# Autodesk Inventor assembly: SensorAssembly_v2
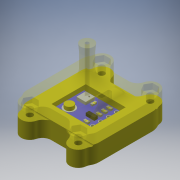
[picture p0: Inventor's stored thumbnail of the model, 180x180]
Saved by Autodesk Inventor 2018 (Build 220112000, 112)
## iProperties
Created: 2020-03-10
Part Number: SensorAssembly_v2
Document SubType Name: Assembly
Designer: Ivan
Author: Ivan
## Documents named in this file (4)
- C:\Users\Ivan\Documents\GitHub\IdealGas\3D Model\SensorAssembly_v2.iam
- C:\Users\Ivan\Documents\GitHub\IdealGas\3D Model\DAQcapsule_v2Bottom.ipt
- C:\Users\Ivan\Documents\GitHub\IdealGas\3D Model\DAQcapsule_v2Top.ipt
- C:\Users\Ivan\Documents\GitHub\IdealGas\3D Model\BMP180.ipt
## Components (3 placed, 3 different names)
1. DAQcapsule_v2Bottom:1 — Mate:1, Mate:4, Mate:5, Angle:1, Mate:6, Mate:7
2. DAQcapsule_v2Top:1 — Mate:1, Mate:6, Mate:7
3. BMP180:1 — Mate:4, Mate:5, Angle:1
## Relationships (6: Mate 5, Angle 1)
- Mate:1: DAQcapsule_v2Bottom:1 ↔ DAQcapsule_v2Top:1
- Mate:4: DAQcapsule_v2Bottom:1 ↔ BMP180:1
- Mate:5: DAQcapsule_v2Bottom:1 ↔ BMP180:1
- Angle:1 (180 deg): DAQcapsule_v2Bottom:1 ↔ BMP180:1
- Mate:6: DAQcapsule_v2Bottom:1 ↔ DAQcapsule_v2Top:1
- Mate:7: DAQcapsule_v2Bottom:1 ↔ DAQcapsule_v2Top:1
